# Autodesk Inventor assembly: connection_6_1
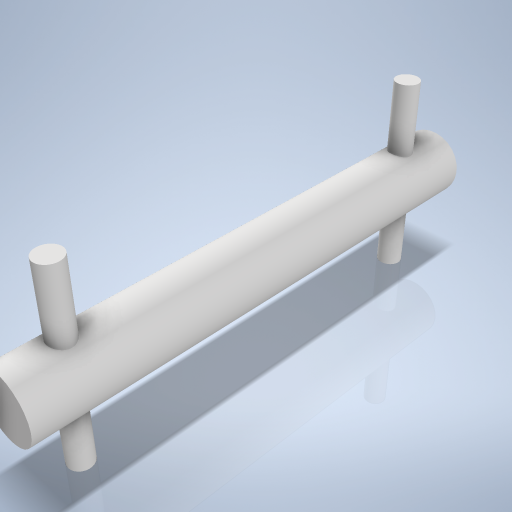
[picture p0: Inventor's stored thumbnail of the model, 512x512]
Saved by Autodesk Inventor 2024.2 (Build 282272000, 272)
## iProperties
Created: 2024-05-05
Part Number: connection_6_1
Document SubType Name: Assembly
Designer: Fabri
Author: Fabri
## Documents named in this file (3)
- C:\Users\Fabri\Documents\Inventor\stirlingEngine\connection_6_1.iam
- C:\Users\Fabri\Documents\Inventor\stirlingEngine\18,1.ipt
- C:\Users\Fabri\Documents\Inventor\stirlingEngine\21.ipt
## Components (3 placed, 2 different names)
1. 18,1:1 — Passend:1, Drehbar:1
2. 18,1:2 — Passend:2, Drehbar:2
3. 21:1 — Passend:1, Passend:2, Drehbar:1, Drehbar:2
## Relationships (4: Mate 2, RevoluteJoint 2)
- Passend:1 [Mate]: 18,1:1 ↔ 21:1
- Passend:2 [Mate]: 18,1:2 ↔ 21:1
- Drehbar:1 [RevoluteJoint] (-30 mm): 18,1:1 ↔ 21:1
- Drehbar:2 [RevoluteJoint] (18 mm): 18,1:2 ↔ 21:1
